# Autodesk Inventor assembly: cam
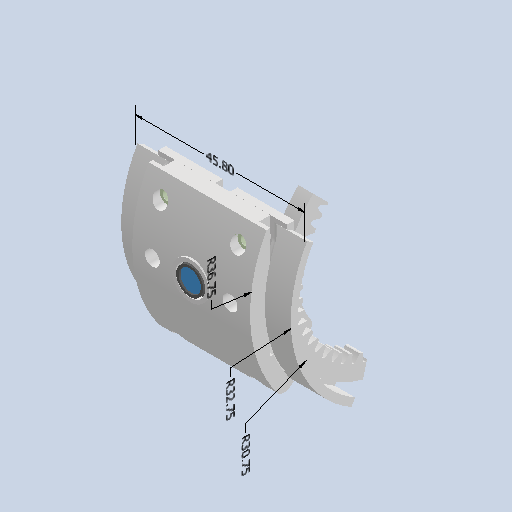
[picture p0: Inventor's stored thumbnail of the model, 512x512]
Saved by Autodesk Inventor 2024.1 (Build 281209000, 209)
## iProperties
Created: 2025-01-10
Part Number: cam
Document SubType Name: Assembly
Designer: hibik
Author: hibik
## Documents named in this file (5)
- C:\Users\hibik\Documents\Robomech\RESCUE\ORCA\hard\camera\cam.iam
- C:\Users\hibik\Documents\Robomech\RESCUE\ORCA\hard\camera\cam.ipt
- C:\Users\hibik\Documents\Robomech\RESCUE\ORCA\hard\camera\cover_front.ipt
- C:\Users\hibik\Documents\Robomech\RESCUE\ORCA\hard\camera\cover_back_right.ipt
- C:\Users\hibik\Documents\Robomech\RESCUE\ORCA\hard\camera\cover_back_left.iam
## Components (4 placed, 4 different names)
1. cam:1 — 挿入:1, 挿入:2, 挿入:3, 挿入:4, 挿入:5, 挿入:6
2. cover_front:1 — 挿入:1, 挿入:2
3. cover_back_right:1 — 挿入:3, 挿入:4
4. cover_back_left:1 [sub-assembly] — 挿入:5, 挿入:6
## Relationships (6: Insert 6)
- 挿入:1 [Insert]: cam:1 ↔ cover_front:1
- 挿入:2 [Insert]: cam:1 ↔ cover_front:1
- 挿入:3 [Insert]: cam:1 ↔ cover_back_right:1
- 挿入:4 [Insert]: cam:1 ↔ cover_back_right:1
- 挿入:5 [Insert]: cam:1 ↔ cover_back_left:1
- 挿入:6 [Insert]: cam:1 ↔ cover_back_left:1
